# Autodesk Inventor assembly: Pressure Vessel, Global Assembly
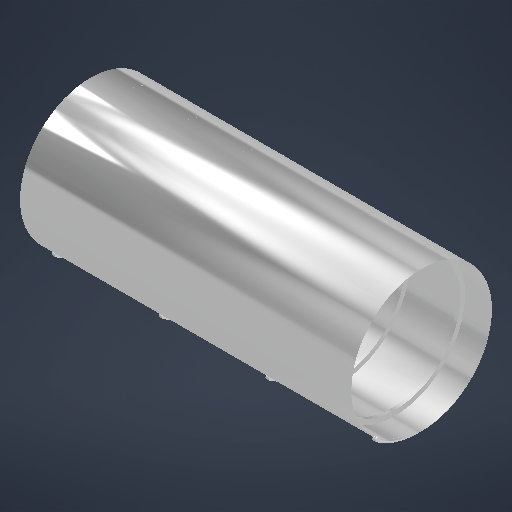
[picture p0: Inventor's stored thumbnail of the model, 512x512]
Saved by Autodesk Inventor 2026 (Build 300175000, 175)
## iProperties
Created: 2025-10-25
Part Number: Pressure Vessel, Global Assembly
Document SubType Name: Assembly
Designer: Brandon Portillo
Mass: 2.22051e+06 g
Surface Area: 3.10148e+06 cm^2
Volume: 890936 cm^3
Density: 2.49233 g/cm^3
Author: Brandon Portillo
## iProperties of the stored document MemberDocs/xRd31mju1Fs0ltyt4Lrp1urqlEg
Created: 2025-10-25
Part Number: Pressure Vessel, Global Assembly
Document SubType Name: Assembly
Designer: Brandon Portillo
Mass: 2.34269e+06 g
Surface Area: 3.3091e+06 cm^2
Volume: 867355 cm^3
Density: 2.70096 g/cm^3
Author: Brandon Portillo
## Documents named in this file (28)
- C:\Users\anarc\GitHub\TSGC-NASA_Senior_Design\CAD\Pressure Vessel\Pressure Vessel, Global Assembly.iam
- C:\Users\anarc\GitHub\TSGC-NASA_Senior_Design\CAD\Pressure Vessel\Pressure Vessel, Single Part.ipt
- C:\Users\anarc\GitHub\TSGC-NASA_Senior_Design\CAD\Pressure Vessel\Saddle.ipt
- C:\Users\anarc\GitHub\TSGC-NASA_Senior_Design\CAD\Pressure Vessel\Support Ring, L-Section.ipt
- C:\Users\anarc\GitHub\TSGC-NASA_Senior_Design\CAD\Pressure Vessel\Floor Frame, I Section.ipt
- C:\Users\anarc\GitHub\TSGC-NASA_Senior_Design\CAD\Pressure Vessel\Floor, Floor.ipt
- C:\Users\anarc\GitHub\TSGC-NASA_Senior_Design\CAD\Pressure Vessel\Floor, Loft.ipt
- C:\Users\anarc\GitHub\TSGC-NASA_Senior_Design\CAD\Pressure Vessel\Water Tank.ipt
- C:\Users\anarc\GitHub\TSGC-NASA_Senior_Design\CAD\Pressure Vessel\Water Tank_MIR.ipt
- C:\Users\anarc\GitHub\TSGC-NASA_Senior_Design\CAD\Pressure Vessel\Floor, Loft_MIR.ipt
- C:\Users\anarc\GitHub\TSGC-NASA_Senior_Design\CAD\Pressure Vessel\Floor, Shower.ipt
- C:\Users\anarc\GitHub\TSGC-NASA_Senior_Design\CAD\Pressure Vessel\Pressure Vessel, Global Assembly\AIP\Cable and Harness\Pressure Vessel, Global Assembly.Harness2.iam
- C:\Users\anarc\GitHub\TSGC-NASA_Senior_Design\CAD\Pressure Vessel\Legs\LegSaddles.iam
- C:\Users\anarc\GitHub\TSGC-NASA_Senior_Design\CAD\Pressure Vessel\Pressure Vessel End Cap\Pressure Vessel Assemble With Door\Pressure Vessel Assemble With Door\Pressure Vessel Assemble With Door.iam
- C:\Users\anarc\GitHub\TSGC-NASA_Senior_Design\CAD\Pressure Vessel\Pressure Vessel, Global Assembly\AIP\FEA\f8hakl7i8.fmsh
- C:\Users\anarc\GitHub\TSGC-NASA_Senior_Design\CAD\Pressure Vessel\Pressure Vessel, Global Assembly\AIP\FEA\f8hakl7i9.fres
- C:\Users\anarc\GitHub\TSGC-NASA_Senior_Design\CAD\Pressure Vessel\Pressure Vessel, Global Assembly\AIP\FEA\f8iu11i74.fins
- C:\Users\anarc\GitHub\TSGC-NASA_Senior_Design\CAD\Pressure Vessel\Pressure Vessel, Global Assembly\AIP\FEA\f8iu11i74.fsat
- C:\Users\anarc\GitHub\TSGC-NASA_Senior_Design\CAD\Pressure Vessel\Pressure Vessel, Global Assembly\AIP\FEA\f8iu11i74.ftes
- C:\Users\anarc\GitHub\TSGC-NASA_Senior_Design\CAD\Pressure Vessel\Pressure Vessel, Global Assembly\AIP\FEA\f8iu11i74.fwiz
- C:\Users\anarc\GitHub\TSGC-NASA_Senior_Design\CAD\Pressure Vessel\Pressure Vessel, Global Assembly\AIP\FEA\f8iu11iao.fmsh
- C:\Users\anarc\GitHub\TSGC-NASA_Senior_Design\CAD\Pressure Vessel\Pressure Vessel, Global Assembly\AIP\FEA\f8iu11iap.fres
- C:\Users\anarc\GitHub\TSGC-NASA_Senior_Design\CAD\Pressure Vessel\Pressure Vessel, Global Assembly\AIP\FEA\f8qf2hwhs.fins
- C:\Users\anarc\GitHub\TSGC-NASA_Senior_Design\CAD\Pressure Vessel\Pressure Vessel, Global Assembly\AIP\FEA\f8qf2hwhs.fsat
- C:\Users\anarc\GitHub\TSGC-NASA_Senior_Design\CAD\Pressure Vessel\Pressure Vessel, Global Assembly\AIP\FEA\f8qf2hwhs.ftes
- C:\Users\anarc\GitHub\TSGC-NASA_Senior_Design\CAD\Pressure Vessel\Pressure Vessel, Global Assembly\AIP\FEA\f8qf2hwhs.fwiz
- C:\Users\anarc\GitHub\TSGC-NASA_Senior_Design\CAD\Pressure Vessel\Pressure Vessel, Global Assembly\AIP\FEA\f8qf2hwqo.fmsh
- C:\Users\anarc\GitHub\TSGC-NASA_Senior_Design\CAD\Pressure Vessel\Pressure Vessel, Global Assembly\AIP\FEA\f8qf2hwrk.fres
## Components (11 placed, 3 different names)
1. Pressure Vessel, Single Part:1 — Mate:8, Flush:15, Tangent:4, Mate:9, Flush:16
2. Saddle:1 — Mate:8, Flush:15
3. Saddle:2
4. Saddle:3
5. Saddle:4
6. Support Ring, L-Section:1 — Mate:9, Flush:16
7. Support Ring, L-Section:2
8. Support Ring, L-Section:3
9. Support Ring, L-Section:4
10. Support Ring, L-Section:5
11. Support Ring, L-Section:6
## Component patterns: (4 elements, first: Saddle:1), (6 elements, first: Support Ring, L-Section:1)
## Relationships (6: Mate 2, Flush 2, Angle 1, Tangent 1)
- Mate:8: Pressure Vessel, Single Part:1 ↔ Saddle:1
- Flush:15 (100 mm): Pressure Vessel, Single Part:1 ↔ Saddle:1
- Angle:3 (0 deg)
- Tangent:4: Pressure Vessel, Single Part:1
- Mate:9: Pressure Vessel, Single Part:1 ↔ Support Ring, L-Section:1
- Flush:16 (800 mm): Pressure Vessel, Single Part:1 ↔ Support Ring, L-Section:1
## Named parameters: sa_0 = 0, sa_1 = -981, sa_2 = 0
note: some values were not read from the file. Shown as the stored number, unit unknown: "sa_0", "sa_1", "sa_2".
